# Autodesk Inventor assembly: Assembly_miniSPIM_v0
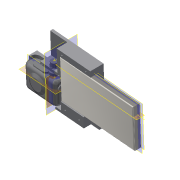
[picture p0: Inventor's stored thumbnail of the model, 180x180]
Saved by Autodesk Inventor 2019 (Build 230136000, 136)
## iProperties
Created: 2019-07-21
Part Number: Assembly_miniSPIM_v0
Document SubType Name: Assembly
Designer: diederichbenedict
Author: diederichbenedict
## Documents named in this file (9)
- C:\Users\diederichbenedict\Dropbox\Dokumente\Promotion\PROJECTS\miniSPIM\INVENTOR\Assembly_miniSPIM_v0.iam
- C:\Users\diederichbenedict\Dropbox\Dokumente\Promotion\PROJECTS\miniSPIM\INVENTOR\100_DXO_Camera v2.ipt
- C:\Users\diederichbenedict\Dropbox\Dokumente\Promotion\PROJECTS\miniSPIM\INVENTOR\101_CCTV_Lens_Thread.ipt
- C:\Users\diederichbenedict\Dropbox\Dokumente\Promotion\PROJECTS\miniSPIM\INVENTOR\103_CCTV_Lens_f2.8_f#1.ipt
- C:\Users\diederichbenedict\Dropbox\Dokumente\Promotion\PROJECTS\miniSPIM\INVENTOR\00_Sony_MDL_Projector.ipt
- C:\Users\diederichbenedict\Dropbox\Dokumente\Promotion\PROJECTS\miniSPIM\INVENTOR\10_Lidplate_Minispim.ipt
- C:\Users\diederichbenedict\Dropbox\Dokumente\Promotion\PROJECTS\miniSPIM\INVENTOR\00_Lens_f_25mm.ipt
- C:\Users\diederichbenedict\Dropbox\Dokumente\Promotion\PROJECTS\miniSPIM\INVENTOR\10_Lid_Minispim.ipt
- C:\Users\diederichbenedict\Dropbox\Dokumente\Promotion\PROJECTS\miniSPIM\INVENTOR\10_Minispim_Base.ipt
## Components (8 placed, 8 different names)
1. 100_DXO_Camera v2:1 — Insert:2, Flush:9, Mate:12, Flush:13
2. 103_CCTV_Lens_f2.8_f#1:1 — Insert:2, Insert:4, Mate:9, Mate:10, Flush:10
3. 101_CCTV_Lens_Thread:2 — Insert:4
4. 10_Lidplate_Minispim:1
5. 00_Lens_f_25mm:1 — Insert:5, Mate:12
6. 10_Lid_Minispim:1
7. 00_Sony_MDL_Projector:1 — Flush:9, Insert:5, Flush:10, Flush:11, Flush:12, Flush:14
8. 10_Minispim_Base:1 — Flush:11, Flush:12, Flush:13, Flush:14
## Relationships (13: Flush 6, Mate 4, Insert 3)
- Insert:2 (-6 mm): 100_DXO_Camera v2:1 ↔ 103_CCTV_Lens_f2.8_f#1:1
- Insert:4 (5 mm): 103_CCTV_Lens_f2.8_f#1:1 ↔ 101_CCTV_Lens_Thread:2
- Mate:9: 103_CCTV_Lens_f2.8_f#1:1
- Mate:10: 103_CCTV_Lens_f2.8_f#1:1
- Mate:11
- Flush:9: 100_DXO_Camera v2:1 ↔ 00_Sony_MDL_Projector:1
- Insert:5 (2 mm): 00_Lens_f_25mm:1 ↔ 00_Sony_MDL_Projector:1
- Mate:12 (17.75 mm): 100_DXO_Camera v2:1 ↔ 00_Lens_f_25mm:1
- Flush:10 (5 mm): 103_CCTV_Lens_f2.8_f#1:1 ↔ 00_Sony_MDL_Projector:1
- Flush:11: 00_Sony_MDL_Projector:1 ↔ 10_Minispim_Base:1
- Flush:12: 00_Sony_MDL_Projector:1 ↔ 10_Minispim_Base:1
- Flush:13: 100_DXO_Camera v2:1 ↔ 10_Minispim_Base:1
- Flush:14: 00_Sony_MDL_Projector:1 ↔ 10_Minispim_Base:1
